# Autodesk Inventor assembly: Gen two arm with body
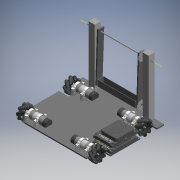
[picture p0: Inventor's stored thumbnail of the model, 180x180]
Saved by Autodesk Inventor 2019 (Build 230136000, 136)
## iProperties
Part Number: Gen two arm with body
Document SubType Name: Assembly
Designer: Delta
Author: Delta
## Documents named in this file (3)
- C:\Robotics\CAD\2019-20_CAD\Collection\Gen two arm with body.iam
- C:\Robotics\CAD\2019-20_CAD\Drive Train\Gen 2.0 Robot.iam
- C:\Robotics\CAD\2019-20_CAD\Collection\Arm for Gen 2.iam
## Components (2 placed, 2 different names)
1. Gen 2.0 Robot:1 [sub-assembly] — Flush:1, Mate:1, Flush:2
2. Arm for Gen 2:1 [sub-assembly] — Flush:1, Mate:1, Flush:2
## Relationships (3: Flush 2, Mate 1)
- Flush:1: Gen 2.0 Robot:1 ↔ Arm for Gen 2:1
- Mate:1: Gen 2.0 Robot:1 ↔ Arm for Gen 2:1
- Flush:2 (63.5 mm): Gen 2.0 Robot:1 ↔ Arm for Gen 2:1
